# Autodesk Inventor assembly: gripper2_v3
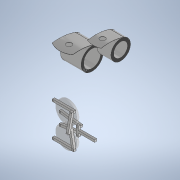
[picture p0: Inventor's stored thumbnail of the model, 180x180]
Saved by Autodesk Inventor 2022 (Build 260153000, 153)
## iProperties
Created: 2022-05-21
Part Number: gripper2_v3
Document SubType Name: Assembly
Designer: kylem
Author: kylem
## Documents named in this file (6)
- C:\Users\kylem\OneDrive\Documents\GitHub\IMML_Contactile_Gripper_Hardware\gripper_v2\gripper2_v3.iam
- C:\Users\kylem\OneDrive\Documents\GitHub\IMML_Contactile_Gripper_Hardware\gripper_v2\drive_shaft.ipt
- C:\Users\kylem\OneDrive\Documents\GitHub\IMML_Contactile_Gripper_Hardware\gripper_v2\drum.ipt
- C:\Users\kylem\OneDrive\Documents\GitHub\IMML_Contactile_Gripper_Hardware\gripper_v2\link.ipt
- C:\Users\kylem\Downloads\9293K117_Constant-Force Spring.ipt
- C:\Users\kylem\Downloads\9293K263_Constant-Force Spring.ipt
## Components (11 placed, 5 different names)
1. drive_shaft:1 — Mate:1, Mate:2, Flush:1, Flush:2, Mate:12, Mate:18, Angle:1, Angle:2
2. drum:1 — Flush:1, Mate:3, Mate:4, Mate:7, Mate:14, Mate:22, Mate:32, Mate:37
3. drum:2 — Flush:2, Mate:5, Mate:6, Mate:9, Mate:13, Mate:21, Mate:31, Mate:36
4. link:1 — Mate:14, Mate:23, Mate:36
5. link:2 — Mate:7, Mate:12, Mate:32
6. link:3 — Mate:9, Mate:18, Mate:31
7. link:4 — Mate:13, Mate:24, Mate:37
8. link:5 — Angle:2, Flush:4, Mate:22, Mate:24
9. link:6 — Angle:1, Flush:3, Mate:21, Mate:23
10. 9293K117_Constant-Force Spring:1
11. 9293K263_Constant-Force Spring:1
## Relationships (26: Mate 20, Flush 4, Angle 2)
- Mate:1: drive_shaft:1
- Mate:2 (-1 mm): drive_shaft:1
- Flush:1: drive_shaft:1 ↔ drum:1
- Mate:3 (10 mm): drum:1
- Mate:4: drum:1
- Flush:2: drive_shaft:1 ↔ drum:2
- Mate:5 (-10 mm): drum:2
- Mate:6: drum:2
- Mate:7: drum:1 ↔ link:2
- Mate:9: drum:2 ↔ link:3
- Mate:12: drive_shaft:1 ↔ link:2
- Mate:13: drum:2 ↔ link:4
- Mate:14 (2 mm): drum:1 ↔ link:1
- Mate:18: drive_shaft:1 ↔ link:3
- Angle:1 (0 deg): drive_shaft:1 ↔ link:6
- Angle:2 (0 deg): drive_shaft:1 ↔ link:5
- Flush:3 (-9 mm): link:6
- Flush:4 (-9 mm): link:5
- Mate:21: drum:2 ↔ link:6
- Mate:22: drum:1 ↔ link:5
- Mate:23: link:1 ↔ link:6
- Mate:24: link:4 ↔ link:5
- Mate:31: drum:2 ↔ link:3
- Mate:32: drum:1 ↔ link:2
- Mate:36: drum:2 ↔ link:1
- Mate:37: drum:1 ↔ link:4
